# Autodesk Inventor assembly: Clam
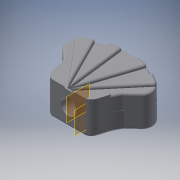
[picture p0: Inventor's stored thumbnail of the model, 180x180]
Saved by Autodesk Inventor 2018 (Build 220112000, 112)
## iProperties
Created: 2018-06-19
Part Number: Clam
Document SubType Name: Assembly
Designer: reide
Author: reide
## Documents named in this file (3)
- C:\Users\reide\OneDrive\Documents\Inventor\TSA\2018\Animatronics\Tortoise\Clam\Clam.iam
- C:\Users\reide\OneDrive\Documents\Inventor\TSA\2018\Animatronics\Tortoise\Clam\ClamPart1v2.ipt
- C:\Users\reide\OneDrive\Documents\Inventor\TSA\2018\Animatronics\Tortoise\Clam\ClamPart2v2.ipt
## Components (2 placed, 2 different names)
1. ClamPart1v2:1 — Mate:1, Mate:2, Mate:3, Flush:2
2. ClamPart2v2:1 — Mate:1, Mate:2, Mate:3, Flush:2
## Relationships (4: Mate 3, Flush 1)
- Mate:1: ClamPart1v2:1 ↔ ClamPart2v2:1
- Mate:2: ClamPart1v2:1 ↔ ClamPart2v2:1
- Mate:3: ClamPart1v2:1 ↔ ClamPart2v2:1
- Flush:2: ClamPart1v2:1 ↔ ClamPart2v2:1
